# Autodesk Inventor assembly: Tire_MIR1
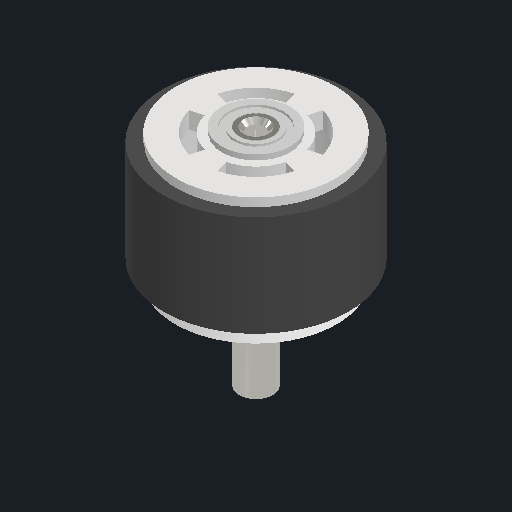
[picture p0: Inventor's stored thumbnail of the model, 512x512]
Saved by Autodesk Inventor 2022 (Build 260153000, 153)
## iProperties
Created: 2021-09-23
Part Number: Tire_MIR1
Document SubType Name: Assembly
Designer: shiok
Author: shiok
## Documents named in this file (7)
- C:\Users\shiok\Documents\GitHub\murakumo\inventor\Tire_MIR1.iam
- C:\Users\shiok\Documents\GitHub\murakumo\inventor\wheel_MIR1.ipt
- C:\Users\shiok\Documents\GitHub\murakumo\inventor\wheelcap_MIR1.ipt
- C:\Users\shiok\Documents\GitHub\murakumo\inventor\Tire_MIR1.ipt
- C:\Users\shiok\Documents\GitHub\murakumo\inventor\spergear_MIR1.ipt
- C:\Users\shiok\Documents\GitHub\murakumo\inventor\FL674ZZ_MIR1.ipt
- C:\Users\shiok\Documents\GitHub\murakumo\inventor\shaft_MIR1.ipt
## Components (8 placed, 6 different names)
1. wheel_MIR1:1 — 挿入:1, 挿入:2, 挿入:3, メイト:1, メイト:5, メイト:4
2. wheelcap_MIR1:1 — 挿入:1, メイト:7, メイト:6
3. Tire_MIR1:1 — 挿入:2
4. spergear_MIR1:1 — 挿入:3, メイト:1, メイト:3, メイト:2
5. FL674ZZ_MIR1:1 — メイト:3, メイト:2
6. FL674ZZ_MIR1:2 — メイト:5, メイト:4
7. FL674ZZ_MIR1:3 — メイト:7, メイト:6, フラッシュ:3, フラッシュ:2, メイト:8, フラッシュ:1
8. shaft_MIR1:1 — フラッシュ:3, フラッシュ:2, メイト:8, フラッシュ:1
## Relationships (14: Mate 8, Insert 3, Flush 3)
- 挿入:1 [Insert]: wheel_MIR1:1 ↔ wheelcap_MIR1:1
- 挿入:2 [Insert]: wheel_MIR1:1 ↔ Tire_MIR1:1
- 挿入:3 [Insert]: wheel_MIR1:1 ↔ spergear_MIR1:1
- メイト:1 [Mate]: wheel_MIR1:1 ↔ spergear_MIR1:1
- メイト:3 [Mate]: spergear_MIR1:1 ↔ FL674ZZ_MIR1:1
- メイト:2 [Mate]: spergear_MIR1:1 ↔ FL674ZZ_MIR1:1
- メイト:5 [Mate]: wheel_MIR1:1 ↔ FL674ZZ_MIR1:2
- メイト:4 [Mate]: wheel_MIR1:1 ↔ FL674ZZ_MIR1:2
- メイト:7 [Mate]: wheelcap_MIR1:1 ↔ FL674ZZ_MIR1:3
- メイト:6 [Mate]: wheelcap_MIR1:1 ↔ FL674ZZ_MIR1:3
- フラッシュ:3 [Flush]: FL674ZZ_MIR1:3 ↔ shaft_MIR1:1
- フラッシュ:2 [Flush]: FL674ZZ_MIR1:3 ↔ shaft_MIR1:1
- メイト:8 [Mate]: FL674ZZ_MIR1:3 ↔ shaft_MIR1:1
- フラッシュ:1 [Flush]: FL674ZZ_MIR1:3 ↔ shaft_MIR1:1
